# Autodesk Inventor assembly: PowerEdge
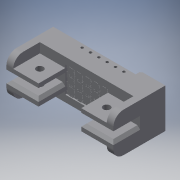
[picture p0: Inventor's stored thumbnail of the model, 180x180]
Saved by Autodesk Inventor 2018 (Build 220112000, 112)
## iProperties
Created: 2017-09-12
Part Number: PowerEdge
Document SubType Name: Assembly
Designer: Srinity
Author: Srinity
## Documents named in this file (3)
- C:\Users\Srinity\Documents\DIY Projects\ModularFRCPlatform\PowerEdge.iam
- C:\Users\Srinity\Documents\DIY Projects\ModularFRCPlatform\Anderson3x5.iam
- C:\Users\Srinity\Documents\DIY Projects\ModularFRCPlatform\AndersonA-BoardEdge.ipt
## Components (2 placed, 2 different names)
1. Anderson3x5:1 [sub-assembly] — Mate:1, Mate:2, Mate:3
2. AndersonA-BoardEdge:1 — Mate:1, Mate:2, Mate:3
## Relationships (3: Mate 3)
- Mate:1: Anderson3x5:1 ↔ AndersonA-BoardEdge:1
- Mate:2: Anderson3x5:1 ↔ AndersonA-BoardEdge:1
- Mate:3: Anderson3x5:1 ↔ AndersonA-BoardEdge:1
